# Autodesk Inventor assembly: Y_Führung
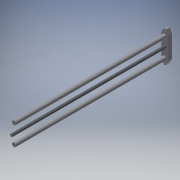
[picture p0: Inventor's stored thumbnail of the model, 180x180]
Saved by Autodesk Inventor 2019 (Build 230136000, 136)
## iProperties
Created: 2018-08-19
Part Number: Y_Führung
Document SubType Name: Assembly
Designer: Julia
Author: Julia
## Documents named in this file (4)
- C:\Users\Julia\Documents\Inventor\3D_Drucker_v01\Y_Führung.iam
- C:\Users\Julia\Documents\Inventor\3D_Drucker_v01\Y_Führungsstange.ipt
- C:\Users\Julia\Documents\Inventor\3D_Drucker_v01\Rahmen_Y_Halterung_v1.ipt
- C:\Users\Julia\Documents\Inventor\3D_Drucker_v01\Gewindestange_Y.ipt
## Components (4 placed, 3 different names)
1. Y_Führungsstange:1 — Mate:1, Mate:4
2. Y_Führungsstange:2 — Mate:3, Mate:5
3. Rahmen_Y_Halterung_v1:1 — Mate:1, Mate:2, Mate:3, Mate:4, Mate:5, Mate:6
4. Gewindestange_Y:1 — Mate:2, Mate:6
## Relationships (6: Mate 6)
- Mate:1: Y_Führungsstange:1 ↔ Rahmen_Y_Halterung_v1:1
- Mate:2: Rahmen_Y_Halterung_v1:1 ↔ Gewindestange_Y:1
- Mate:3: Y_Führungsstange:2 ↔ Rahmen_Y_Halterung_v1:1
- Mate:4: Y_Führungsstange:1 ↔ Rahmen_Y_Halterung_v1:1
- Mate:5: Y_Führungsstange:2 ↔ Rahmen_Y_Halterung_v1:1
- Mate:6: Rahmen_Y_Halterung_v1:1 ↔ Gewindestange_Y:1
